# Autodesk Inventor assembly: Waist-Chest
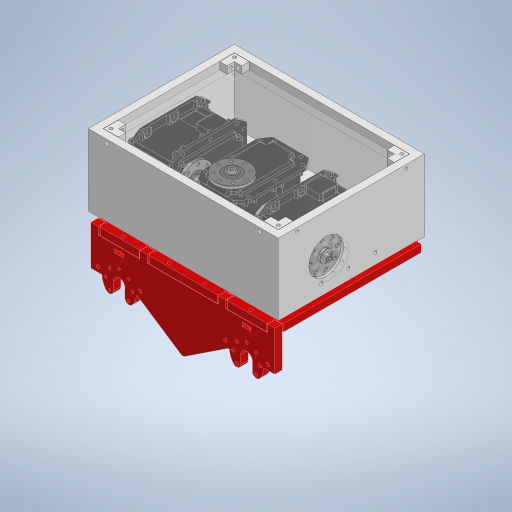
[picture p0: Inventor's stored thumbnail of the model, 512x512]
Saved by Autodesk Inventor 2024 (Build 280153000, 153)
## iProperties
Created: 2024-09-18
Part Number: Waist-Chest
Document SubType Name: Assembly
Designer: Eungang
Author: Eungang
## Documents named in this file (12)
- C:\Users\Eungang\Documents\Inventor\FIGHTING_ROBOT_FINAL\부품\Waist-Chest\Waist.iam
- C:\Users\Eungang\Documents\Inventor\FIGHTING_ROBOT_FINAL\부품\Waist-Chest\pants.ipt
- C:\Users\Eungang\Documents\Inventor\FIGHTING_ROBOT_FINAL\부품\Waist-Chest\waist.ipt
- C:\Users\Eungang\Documents\Inventor\FIGHTING_ROBOT_FINAL\부품\혼\64-106Horn.ipt
- C:\Users\Eungang\Documents\Inventor\FIGHTING_ROBOT_FINAL\부품\아이들러\64아이들러.iam
- C:\Users\Eungang\Documents\Inventor\FIGHTING_ROBOT_FINAL\부품\Waist-Chest\64horn.ipt
- C:\Users\Eungang\Documents\Inventor\FIGHTING_ROBOT_FINAL\부품\Waist-Chest\chest.ipt
- C:\Users\Eungang\Documents\Inventor\FIGHTING_ROBOT_FINAL\부품\Waist-Chest\chest_box_cap.ipt
- C:\Users\Eungang\Documents\Inventor\FIGHTING_ROBOT_FINAL\부품\Waist-Chest\chest_box_cap_connect.ipt
- C:\Users\Eungang\Documents\Inventor\FIGHTING_ROBOT_FINAL\부품\Bolt_Washer_Nut\CSH-STN-M3-8_203.ipt
- C:\Users\Eungang\Documents\Inventor\FIGHTING_ROBOT_FINAL\부품\Bolt_Washer_Nut\CSH-ST-M2_5-15_203.ipt
- C:\Users\Eungang\Documents\Inventor\FIGHTING_ROBOT_FINAL\부품\다이나믹셀\MX-64T.ipt
## Components (34 placed, 11 different names)
1. waist:1 — 메이트:1, 메이트:2, 메이트:3, 메이트:4, 삽입:16, 각도:1, 삽입:41, 삽입:42, 삽입:43, 삽입:44, 삽입:45, 삽입:46, 삽입:47, 삽입:48
2. pants:1 — 메이트:2, 메이트:3, 메이트:4
3. 64horn_extension:1 — 삽입:16, 삽입:23, 삽입:34
4. 64-106Horn:3 — 삽입:23, 삽입:34, 삽입:37, 삽입:56
5. 64아이들러:4 [sub-assembly] — 삽입:38
6. 64-106Horn:4 — 삽입:26, 삽입:32, 삽입:35
7. 64아이들러:5 [sub-assembly] — 삽입:39
8. 64-106Horn:5 — 삽입:29, 삽입:33, 삽입:36
9. 64아이들러:6 [sub-assembly] — 삽입:40
10. chest:1 — 메이트:13, 메이트:15, 메이트:16, 메이트:18, 메이트:19, 메이트:20, 삽입:30, 각도:1, 삽입:51, 삽입:52, 삽입:53, 삽입:54, 삽입:55, 삽입:57, 삽입:58, 삽입:59, 삽입:60
11. 64horn_extension:2 — 삽입:26, 삽입:32
12. chest_box_cap_connect:1 — 삽입:30, 삽입:52
13. chest_box_cap_connect:2 — 메이트:13, 메이트:15, 삽입:62
14. chest_box_cap_connect:3 — 메이트:19, 메이트:20, 삽입:51
15. chest_box_cap_connect:4 — 메이트:16, 메이트:18, 삽입:53, 삽입:61
16. 64horn_extension:3 — 삽입:29, 삽입:33
17. CSH-STN-M3-8_203:1 — 삽입:36
18. CSH-STN-M3-8_203:2 — 삽입:35
19. CSH-STN-M3-8_203:3 — 삽입:37
20. CSH-STN-M3-8_203:4 — 삽입:40
21. CSH-STN-M3-8_203:5 — 삽입:39
22. CSH-STN-M3-8_203:6 — 삽입:38
23. CSH-ST-M2_5-15_203:2 — 삽입:41
24. CSH-ST-M2_5-15_203:3 — 삽입:47
25. CSH-ST-M2_5-15_203:4 — 삽입:46
26. CSH-ST-M2_5-15_203:5 — 삽입:45
27. CSH-ST-M2_5-15_203:6 — 삽입:44
28. CSH-ST-M2_5-15_203:7 — 삽입:43
29. CSH-ST-M2_5-15_203:8 — 삽입:42
30. CSH-ST-M2_5-15_203:9 — 삽입:48
31. MX-64T:1 — 삽입:54, 삽입:55
32. MX-64T:2 — 삽입:56, 삽입:57, 삽입:58
33. chest_box_cap:1 — 삽입:61, 삽입:62
34. MX-64T:3 — 삽입:59, 삽입:60
## Relationships (45: Insert 34, Mate 10, Angle 1)
- 메이트:1 [Mate]: waist:1
- 메이트:2 [Mate] (0.2 mm): waist:1 ↔ pants:1
- 메이트:3 [Mate] (0.2 mm): waist:1 ↔ pants:1
- 메이트:4 [Mate] (0.2 mm): waist:1 ↔ pants:1
- 삽입:16 [Insert]: waist:1 ↔ 64horn_extension:1
- 삽입:23 [Insert]: 64horn_extension:1 ↔ 64-106Horn:3
- 삽입:26 [Insert]: 64-106Horn:4 ↔ 64horn_extension:2
- 메이트:13 [Mate] (0.2 mm): chest:1 ↔ chest_box_cap_connect:2
- 메이트:15 [Mate] (0.2 mm): chest:1 ↔ chest_box_cap_connect:2
- 메이트:16 [Mate] (0.2 mm): chest:1 ↔ chest_box_cap_connect:4
- 메이트:18 [Mate] (0.2 mm): chest:1 ↔ chest_box_cap_connect:4
- 메이트:19 [Mate] (0.2 mm): chest:1 ↔ chest_box_cap_connect:3
- 메이트:20 [Mate] (0.2 mm): chest:1 ↔ chest_box_cap_connect:3
- 삽입:29 [Insert]: 64-106Horn:5 ↔ 64horn_extension:3
- 삽입:30 [Insert] (0.2 mm): chest:1 ↔ chest_box_cap_connect:1
- 각도:1 [Angle] (0 deg): waist:1 ↔ chest:1
- 삽입:32 [Insert]: 64-106Horn:4 ↔ 64horn_extension:2
- 삽입:33 [Insert]: 64-106Horn:5 ↔ 64horn_extension:3
- 삽입:34 [Insert]: 64horn_extension:1 ↔ 64-106Horn:3
- 삽입:35 [Insert]: 64-106Horn:4 ↔ CSH-STN-M3-8_203:2
- 삽입:36 [Insert]: 64-106Horn:5 ↔ CSH-STN-M3-8_203:1
- 삽입:37 [Insert]: 64-106Horn:3 ↔ CSH-STN-M3-8_203:3
- 삽입:38 [Insert]: 64아이들러:4 ↔ CSH-STN-M3-8_203:6
- 삽입:39 [Insert]: 64아이들러:5 ↔ CSH-STN-M3-8_203:5
- 삽입:40 [Insert]: 64아이들러:6 ↔ CSH-STN-M3-8_203:4
- 삽입:41 [Insert]: waist:1 ↔ CSH-ST-M2_5-15_203:2
- 삽입:42 [Insert]: waist:1 ↔ CSH-ST-M2_5-15_203:8
- 삽입:43 [Insert]: waist:1 ↔ CSH-ST-M2_5-15_203:7
- 삽입:44 [Insert]: waist:1 ↔ CSH-ST-M2_5-15_203:6
- 삽입:45 [Insert]: waist:1 ↔ CSH-ST-M2_5-15_203:5
- 삽입:46 [Insert]: waist:1 ↔ CSH-ST-M2_5-15_203:4
- 삽입:47 [Insert]: waist:1 ↔ CSH-ST-M2_5-15_203:3
- 삽입:48 [Insert]: waist:1 ↔ CSH-ST-M2_5-15_203:9
- 삽입:51 [Insert] (0.2 mm): chest:1 ↔ chest_box_cap_connect:3
- 삽입:52 [Insert] (0.2 mm): chest:1 ↔ chest_box_cap_connect:1
- 삽입:53 [Insert] (0.2 mm): chest:1 ↔ chest_box_cap_connect:4
- 삽입:54 [Insert] (0.2 mm): chest:1 ↔ MX-64T:1
- 삽입:55 [Insert] (0.2 mm): chest:1 ↔ MX-64T:1
- 삽입:56 [Insert] (0.5 mm): 64-106Horn:3 ↔ MX-64T:2
- 삽입:57 [Insert]: chest:1 ↔ MX-64T:2
- 삽입:58 [Insert]: chest:1 ↔ MX-64T:2
- 삽입:59 [Insert] (0.2 mm): chest:1 ↔ MX-64T:3
- 삽입:60 [Insert] (0.2 mm): chest:1 ↔ MX-64T:3
- 삽입:61 [Insert]: chest_box_cap_connect:4 ↔ chest_box_cap:1
- 삽입:62 [Insert]: chest_box_cap_connect:2 ↔ chest_box_cap:1
